# Autodesk Inventor assembly: колеса
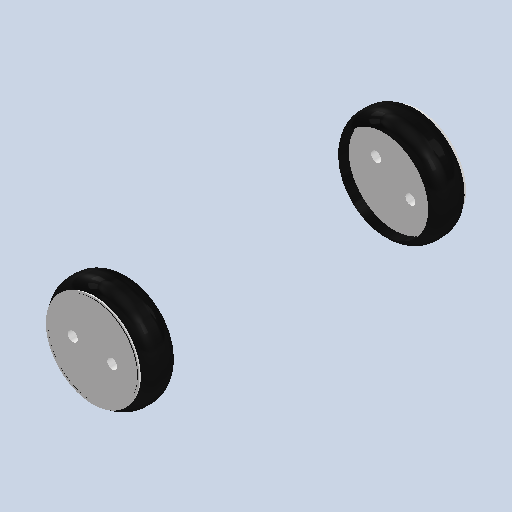
[picture p0: Inventor's stored thumbnail of the model, 512x512]
Saved by Autodesk Inventor 2022 (Build 260153000, 153)
## iProperties
Created: 2025-02-02
Part Number: колеса
Document SubType Name: Assembly
Designer: Admin
Author: Admin
## Documents named in this file (3)
- G:\машина\колеса.iam
- G:\машина\диск заднего колеса.ipt
- G:\машина\шина.ipt
## Components (4 placed, 2 different names)
1. диск заднего колеса:1
2. диск заднего колеса:2
3. шина:1
4. шина:2
## Relationships (4: Mate 4)
- [Mate]: диск заднего колеса:2 ↔ шина:1
- [Mate]: диск заднего колеса:1 ↔ шина:2
- [Mate]: диск заднего колеса:2 ↔ шина:1
- [Mate]: диск заднего колеса:1 ↔ шина:2
